# Autodesk Inventor assembly: weld
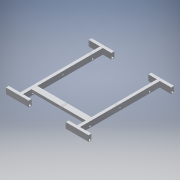
[picture p0: Inventor's stored thumbnail of the model, 180x180]
Saved by Autodesk Inventor 2016 (Build 200138000, 138)
## iProperties
Created: 2016-01-18
Part Number: weld
Document SubType Name: Assembly
Designer: gus
Author: gus
## Documents named in this file (4)
- \\Mac\Home\Desktop\1510-stronghold-CAD\weld\weld.iam
- \\Mac\Home\Desktop\1510-stronghold-CAD\weld\1x2x8in.ipt
- \\Mac\Home\Desktop\1510-stronghold-CAD\weld\1x2x19.ipt
- \\Mac\Home\Desktop\1510-stronghold-CAD\weld\1x2x28.ipt
## Components (7 placed, 3 different names)
1. 1x2x8in:1 — Flush:8, Mate:9, Flush:9, Flush:10
2. 1x2x19:1 — Flush:13, Mate:10, Flush:14, Flush:15, Mate:11, Mate:12
3. 1x2x28:1 — Mate:2, Flush:2, Flush:5, Mate:8, Flush:7, Flush:11, Mate:10, Flush:14
4. 1x2x8in:2 — Mate:8, Flush:7, Flush:11, Flush:12, Mate:12
5. 1x2x8in:3 — Mate:1, Flush:1, Flush:10
6. 1x2x8in:4 — Mate:2, Flush:2, Flush:12
7. 1x2x28:2 — Mate:1, Flush:1, Flush:5, Flush:8, Mate:9, Flush:9, Flush:13, Flush:15, Mate:11
## Relationships (19: Flush 12, Mate 7)
- Mate:1: 1x2x8in:3 ↔ 1x2x28:2
- Flush:1: 1x2x8in:3 ↔ 1x2x28:2
- Mate:2: 1x2x28:1 ↔ 1x2x8in:4
- Flush:2: 1x2x28:1 ↔ 1x2x8in:4
- Flush:5: 1x2x28:1 ↔ 1x2x28:2
- Mate:8: 1x2x28:1 ↔ 1x2x8in:2
- Flush:7: 1x2x28:1 ↔ 1x2x8in:2
- Flush:8: 1x2x8in:1 ↔ 1x2x28:2
- Mate:9: 1x2x8in:1 ↔ 1x2x28:2
- Flush:9 (76.2 mm): 1x2x8in:1 ↔ 1x2x28:2
- Flush:10: 1x2x8in:1 ↔ 1x2x8in:3
- Flush:11 (-76.2 mm): 1x2x28:1 ↔ 1x2x8in:2
- Flush:12: 1x2x8in:2 ↔ 1x2x8in:4
- Flush:13: 1x2x19:1 ↔ 1x2x28:2
- Mate:10: 1x2x19:1 ↔ 1x2x28:1
- Flush:14: 1x2x19:1 ↔ 1x2x28:1
- Flush:15: 1x2x19:1 ↔ 1x2x28:2
- Mate:11: 1x2x19:1 ↔ 1x2x28:2
- Mate:12 (76.2 mm): 1x2x19:1 ↔ 1x2x8in:2
